# Autodesk Inventor assembly: TempController
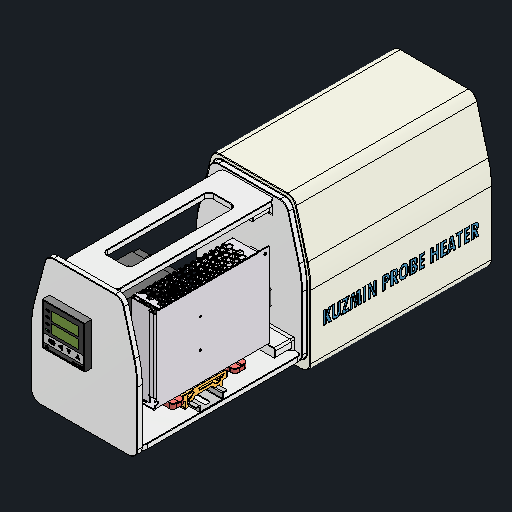
[picture p0: Inventor's stored thumbnail of the model, 512x512]
Saved by Autodesk Inventor 2027.1 (Build 311270010, 270A)
## iProperties
Created: 2025-05-30
Part Number: TempController
Document SubType Name: Assembly
Designer: kuzmin
Author: kuzmin
## Documents named in this file (13)
- C:\Users\queezz\Dropbox\Drawings\PIHTI\ElectronicsBox\TempController\TempController.iam
- C:\Users\queezz\Dropbox\Drawings\PIHTI\ElectronicsBox\TempController\RKC CONTROLLER.ipt
- C:\Users\queezz\Dropbox\Drawings\PIHTI\ElectronicsBox\TempController\Fuente meanwell LRS-100-12.ipt
- C:\Users\queezz\Dropbox\Drawings\PIHTI\ElectronicsBox\TempController\tc-front-panel.ipt
- C:\Users\queezz\Dropbox\Drawings\PIHTI\ElectronicsBox\TempController\RT-65D-Bracket TempController.ipt
- C:\Users\queezz\Dropbox\Drawings\PIHTI\ElectronicsBox\TempController\DIN-rail-tc.ipt
- C:\Users\queezz\Dropbox\Drawings\PIHTI\ElectronicsBox\TempController\tc-bottom-tray.ipt
- C:\Users\queezz\Dropbox\Drawings\PIHTI\ElectronicsBox\TempController\SSR-on-DIN backup.iam
- C:\Users\queezz\Dropbox\Drawings\PIHTI\ElectronicsBox\TempController\IEC320 C14 Panel switch.ipt
- C:\Users\queezz\Dropbox\Drawings\PIHTI\ElectronicsBox\TempController\tc-back-panel.ipt
- C:\Users\queezz\Dropbox\Drawings\PIHTI\ElectronicsBox\TempController\tc-case.ipt
- C:\Users\queezz\Dropbox\Drawings\PIHTI\ElectronicsBox\TempController\tc-top-bar.ipt
- C:\Users\queezz\Dropbox\Drawings\PIHTI\ElectronicsBox\TempController\Wide Din Clip V1.ipt
## Components (12 placed, 12 different names)
1. tc-front-panel:1 — Mate:1, Mate:2, Mate:3, Mate:7, Flush:1, Flush:3, Flush:4, Flush:5, Flush:6, Mate:14, Flush:8
2. RKC CONTROLLER:1 — Mate:1, Mate:2, Mate:3
3. Fuente meanwell LRS-100-12:1 — Rigid:1
4. RT-65D-Bracket:1 — Rigid:1, Rigid:2
5. DIN-rail-tc:1 — Mate:6, Flush:2, Mate:8, Mate:9, Mate:17, Mate:18
6. tc-bottom-tray:1 — Mate:6, Mate:7, Flush:1, Flush:2, Flush:3, Mate:10
7. SSR-on-DIN:1 [sub-assembly] — Mate:8, Mate:9
8. IEC320 C14 Panel switch:1 — Mate:11, Mate:12, Mate:13
9. tc-back-panel:1 — Flush:4, Flush:5, Mate:10, Mate:11, Mate:12, Mate:13, Mate:15, Mate:16, Flush:9
10. tc-case:1 — Flush:6, Mate:14, Mate:15
11. tc-top-bar:1 — Mate:16, Flush:7, Flush:9
12. Wide Din Clip V1:1 — Rigid:2, Mate:17, Mate:18
## Relationships (27: Mate 16, Flush 9, WeldJoint 2)
- Mate:1: tc-front-panel:1 ↔ RKC CONTROLLER:1
- Mate:2: tc-front-panel:1 ↔ RKC CONTROLLER:1
- Mate:3: tc-front-panel:1 ↔ RKC CONTROLLER:1
- Rigid:1 [WeldJoint]: Fuente meanwell LRS-100-12:1 ↔ RT-65D-Bracket:1
- Mate:6: DIN-rail-tc:1 ↔ tc-bottom-tray:1
- Mate:7: tc-front-panel:1 ↔ tc-bottom-tray:1
- Flush:1: tc-front-panel:1 ↔ tc-bottom-tray:1
- Flush:2: DIN-rail-tc:1 ↔ tc-bottom-tray:1
- Flush:3 (5 mm): tc-front-panel:1 ↔ tc-bottom-tray:1
- Mate:8: DIN-rail-tc:1 ↔ SSR-on-DIN:1
- Mate:9: DIN-rail-tc:1 ↔ SSR-on-DIN:1
- Flush:4: tc-front-panel:1 ↔ tc-back-panel:1
- Flush:5: tc-front-panel:1 ↔ tc-back-panel:1
- Mate:10: tc-bottom-tray:1 ↔ tc-back-panel:1
- Mate:11: IEC320 C14 Panel switch:1 ↔ tc-back-panel:1
- Mate:12: IEC320 C14 Panel switch:1 ↔ tc-back-panel:1
- Mate:13: IEC320 C14 Panel switch:1 ↔ tc-back-panel:1
- Flush:6: tc-front-panel:1 ↔ tc-case:1
- Mate:14: tc-front-panel:1 ↔ tc-case:1
- Mate:15: tc-back-panel:1 ↔ tc-case:1
- Mate:16: tc-back-panel:1 ↔ tc-top-bar:1
- Flush:7: tc-top-bar:1
- Flush:8: tc-front-panel:1
- Flush:9 (2 mm): tc-back-panel:1 ↔ tc-top-bar:1
- Rigid:2 [WeldJoint]: RT-65D-Bracket:1 ↔ Wide Din Clip V1:1
- Mate:17: DIN-rail-tc:1 ↔ Wide Din Clip V1:1
- Mate:18: DIN-rail-tc:1 ↔ Wide Din Clip V1:1
